# Autodesk Inventor assembly: Team24_Assembly_Fixed
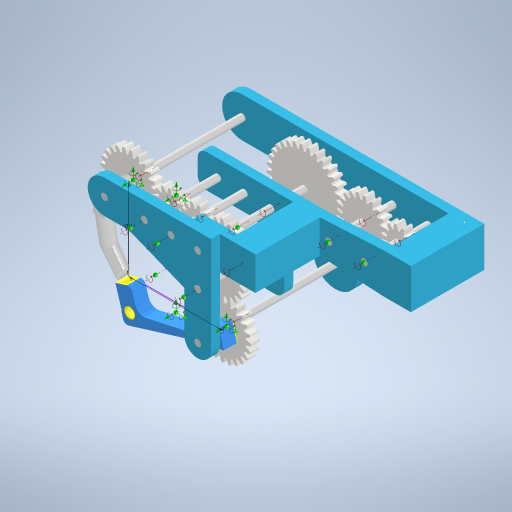
[picture p0: Inventor's stored thumbnail of the model, 512x512]
Saved by Autodesk Inventor 2024 (Build 280153000, 153)
## iProperties
Created: 2024-01-19
Part Number: Team24_Assembly_Fixed
Document SubType Name: Assembly
Designer: clbri
Author: clbri
## Documents named in this file (13)
- C:\Users\clbri\Downloads\Team24_MM9\Team24_Assembly_Fixed.iam
- C:\Users\clbri\Downloads\Team24_MM9\Mounting Bracket Files\bridgc1_MountingBracket_1of3_Modified.ipt
- C:\Users\clbri\Downloads\Team24_MM9\Mounting Bracket Files\bridgc1_MountingBracket_3of3_Modified.ipt
- C:\Users\clbri\Downloads\Team24_MM9\Mounting Bracket Files\bridgc1_MountingBracket_2of3_Modified.ipt
- C:\Users\clbri\Downloads\Team24_MM9\Mounting Bracket Files\Rod_66mm.ipt
- C:\Users\clbri\Downloads\Team24_MM9\Mounting Bracket Files\Rod_37mm.ipt
- C:\Users\clbri\Downloads\Team24_MM9\Gears\IO_Gear (z=12).ipt
- C:\Users\clbri\Downloads\Team24_MM9\Gears\IO_Gear (z=20).ipt
- C:\Users\clbri\Downloads\Team24_MM9\Gears\IO_Gear (z=32).ipt
- C:\Users\clbri\Downloads\Team24_MM9\Gears\IO_Gear (z=24).ipt
- C:\Users\clbri\Downloads\Team24_MM9\Gears\IdlerGear (z=18).ipt
- C:\Users\clbri\Downloads\Team24_MM9\Forefinger and Thumb\bridgc1_Forefinger (2).ipt
- C:\Users\clbri\Downloads\Team24_MM9\Forefinger and Thumb\mohsis8_thumb.ipt
## Components (22 placed, 12 different names)
1. bridgc1_MountingBracket_1of3_Modified:1 — Flush:1, Flush:2, Mate:1, Mate:21
2. bridgc1_MountingBracket_3of3_Modified:1 — Flush:1, Flush:2, Mate:1, Mate:2, Flush:3, Flush:4, Mate:3, Mate:4, Flush:9, Flush:10, Mate:9, Angle:1
3. bridgc1_MountingBracket_2of3_Modified:1 — Mate:2, Flush:3, Flush:4, Mate:5, Mate:7, Mate:8, Flush:5, Flush:6, Flush:7, Mate:10, Flush:11, Flush:12, Mate:11, Flush:13, Mate:22, Angle:2, Angle:3
4. Rod_66mm:1 — Mate:10, Flush:11, Mate:18, Mate:23, Mate:32, Mate:35
5. Rod_66mm:2 — Mate:9, Flush:12, Mate:15, Mate:17, Mate:26, Mate:27
6. Rod_37mm:1 — Mate:4, Flush:10, Mate:16, Mate:28
7. Rod_37mm:2 — Mate:3, Flush:9, Mate:12, Mate:29
8. Rod_37mm:3 — Mate:5, Flush:7, Mate:19, Mate:30
9. Rod_37mm:4 — Mate:8, Flush:5, Mate:14, Mate:24
10. Rod_37mm:5 — Mate:7, Flush:6, Mate:13, Mate:25
11. Rod_66mm:3 — Mate:11, Flush:13, Mate:20, Mate:31, Mate:36, Angle:2, Angle:4
12. IO_Gear (z=12):1 — Mate:15, Flush:17, Flush:18, Mate:27
13. IO_Gear (z=12):2 — Mate:13, Flush:16, Flush:17, Mate:25
14. IO_Gear (z=12):3 — Mate:12, Flush:15, Mate:29
15. IO_Gear (z=12):4 — Mate:14, Mate:22, Flush:16, Flush:20, Mate:24
16. IO_Gear (z=20):1 — Mate:16, Flush:14, Flush:15, Mate:28
17. IO_Gear (z=32):1 — Mate:17, Mate:21, Flush:14, Mate:26
18. IO_Gear (z=24):1 — Mate:20, Flush:19, Mate:31, Mate:37
19. IO_Gear (z=24):2 — Mate:18, Flush:20, Mate:23, Mate:33
20. IdlerGear (z=18):1 — Mate:19, Flush:18, Flush:19, Mate:30
21. bridgc1_Forefinger (2):1 — Mate:32, Mate:33, Mate:35, Angle:1
22. mohsis8_thumb:1 — Mate:36, Mate:37, Angle:3, Angle:4
## Relationships (58: Mate 35, Flush 19, Angle 4)
- Flush:1: bridgc1_MountingBracket_1of3_Modified:1 ↔ bridgc1_MountingBracket_3of3_Modified:1
- Flush:2: bridgc1_MountingBracket_1of3_Modified:1 ↔ bridgc1_MountingBracket_3of3_Modified:1
- Mate:1: bridgc1_MountingBracket_1of3_Modified:1 ↔ bridgc1_MountingBracket_3of3_Modified:1
- Mate:2: bridgc1_MountingBracket_3of3_Modified:1 ↔ bridgc1_MountingBracket_2of3_Modified:1
- Flush:3: bridgc1_MountingBracket_3of3_Modified:1 ↔ bridgc1_MountingBracket_2of3_Modified:1
- Flush:4: bridgc1_MountingBracket_3of3_Modified:1 ↔ bridgc1_MountingBracket_2of3_Modified:1
- Mate:3: bridgc1_MountingBracket_3of3_Modified:1 ↔ Rod_37mm:2
- Mate:4: bridgc1_MountingBracket_3of3_Modified:1 ↔ Rod_37mm:1
- Mate:5: bridgc1_MountingBracket_2of3_Modified:1 ↔ Rod_37mm:3
- Mate:7: bridgc1_MountingBracket_2of3_Modified:1 ↔ Rod_37mm:5
- Mate:8: bridgc1_MountingBracket_2of3_Modified:1 ↔ Rod_37mm:4
- Flush:5: bridgc1_MountingBracket_2of3_Modified:1 ↔ Rod_37mm:4
- Flush:6: bridgc1_MountingBracket_2of3_Modified:1 ↔ Rod_37mm:5
- Flush:7: bridgc1_MountingBracket_2of3_Modified:1 ↔ Rod_37mm:3
- Flush:9: bridgc1_MountingBracket_3of3_Modified:1 ↔ Rod_37mm:2
- Flush:10: bridgc1_MountingBracket_3of3_Modified:1 ↔ Rod_37mm:1
- Mate:9: bridgc1_MountingBracket_3of3_Modified:1 ↔ Rod_66mm:2
- Mate:10: bridgc1_MountingBracket_2of3_Modified:1 ↔ Rod_66mm:1
- Flush:11: bridgc1_MountingBracket_2of3_Modified:1 ↔ Rod_66mm:1
- Flush:12: bridgc1_MountingBracket_2of3_Modified:1 ↔ Rod_66mm:2
- Mate:11: bridgc1_MountingBracket_2of3_Modified:1 ↔ Rod_66mm:3
- Flush:13: bridgc1_MountingBracket_2of3_Modified:1 ↔ Rod_66mm:3
- Mate:12: Rod_37mm:2 ↔ IO_Gear (z=12):3
- Mate:13: Rod_37mm:5 ↔ IO_Gear (z=12):2
- Mate:14: Rod_37mm:4 ↔ IO_Gear (z=12):4
- Mate:15: Rod_66mm:2 ↔ IO_Gear (z=12):1
- Mate:16: Rod_37mm:1 ↔ IO_Gear (z=20):1
- Mate:17: Rod_66mm:2 ↔ IO_Gear (z=32):1
- Mate:18: Rod_66mm:1 ↔ IO_Gear (z=24):2
- Mate:19: Rod_37mm:3 ↔ IdlerGear (z=18):1
- Mate:20: Rod_66mm:3 ↔ IO_Gear (z=24):1
- Mate:21 (10 mm): bridgc1_MountingBracket_1of3_Modified:1 ↔ IO_Gear (z=32):1
- Flush:14: IO_Gear (z=20):1 ↔ IO_Gear (z=32):1
- Flush:15: IO_Gear (z=12):3 ↔ IO_Gear (z=20):1
- Mate:22 (7 mm): bridgc1_MountingBracket_2of3_Modified:1 ↔ IO_Gear (z=12):4
- Flush:16: IO_Gear (z=12):2 ↔ IO_Gear (z=12):4
- Flush:17: IO_Gear (z=12):1 ↔ IO_Gear (z=12):2
- Flush:18: IO_Gear (z=12):1 ↔ IdlerGear (z=18):1
- Flush:19: IO_Gear (z=24):1 ↔ IdlerGear (z=18):1
- Flush:20: IO_Gear (z=12):4 ↔ IO_Gear (z=24):2
- Mate:23: Rod_66mm:1 ↔ IO_Gear (z=24):2
- Mate:24: Rod_37mm:4 ↔ IO_Gear (z=12):4
- Mate:25: Rod_37mm:5 ↔ IO_Gear (z=12):2
- Mate:26: Rod_66mm:2 ↔ IO_Gear (z=32):1
- Mate:27: Rod_66mm:2 ↔ IO_Gear (z=12):1
- Mate:28: Rod_37mm:1 ↔ IO_Gear (z=20):1
- Mate:29: Rod_37mm:2 ↔ IO_Gear (z=12):3
- Mate:30: Rod_37mm:3 ↔ IdlerGear (z=18):1
- Mate:31: Rod_66mm:3 ↔ IO_Gear (z=24):1
- Mate:32: Rod_66mm:1 ↔ bridgc1_Forefinger (2):1
- Mate:33: IO_Gear (z=24):2 ↔ bridgc1_Forefinger (2):1
- Mate:35: Rod_66mm:1 ↔ bridgc1_Forefinger (2):1
- Mate:36: Rod_66mm:3 ↔ mohsis8_thumb:1
- Mate:37: IO_Gear (z=24):1 ↔ mohsis8_thumb:1
- Angle:1 (0 deg): bridgc1_MountingBracket_3of3_Modified:1 ↔ bridgc1_Forefinger (2):1
- Angle:2 (0 deg): bridgc1_MountingBracket_2of3_Modified:1 ↔ Rod_66mm:3
- Angle:3 (-17 deg): bridgc1_MountingBracket_2of3_Modified:1 ↔ mohsis8_thumb:1
- Angle:4 (0 deg): Rod_66mm:3 ↔ mohsis8_thumb:1
